# Autodesk Inventor assembly: КВ33.044.400 - Сборка деражтеля катка 6 мм
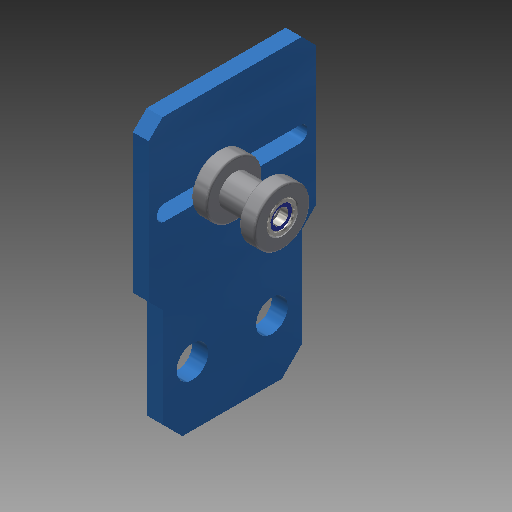
[picture p0: Inventor's stored thumbnail of the model, 512x512]
Saved by Autodesk Inventor 2019 (Build 230136000, 136)
## iProperties
Created: 2019-07-17
Part Number: КВ33.044.400 - Сборка деражтеля катка 6 мм
Material: Типовые
Document SubType Name: Assembly
Designer: Петров Иван
Mass: 12.6725 g
Surface Area: 80.5555 cm^2
Volume: 11.4117 cm^3
Density: 1.11049 g/cm^3
Author: Петров Иван
## Documents named in this file (3)
- E:\IVAN\Ivan_desktop\Kvantorium\Projects\optimal_gripper\hardware\КВ33.044.800 - Сборка держателя катка.iam
- E:\IVAN\Ivan_desktop\Kvantorium\Projects\optimal_gripper\hardware\КВ33.044.801 - Держатель катка.ipt
- E:\IVAN\Ivan_desktop\Kvantorium\Projects\optimal_gripper\hardware\Стандартные изделия\Шкив плоский Makeblock сборка.iam
## Components (2 placed, 2 different names)
1. КВ33.044.801 - Держатель катка:1 — Совмещение:1, Касательность:1
2. Шкив плоский Makeblock сборка:1 [sub-assembly] — Совмещение:1, Касательность:1
## Relationships (2: Mate 1, Tangent 1)
- Совмещение:1 [Mate]: КВ33.044.801 - Держатель катка:1 ↔ Шкив плоский Makeblock сборка:1
- Касательность:1 [Tangent]: КВ33.044.801 - Держатель катка:1 ↔ Шкив плоский Makeblock сборка:1
